# Autodesk Inventor assembly: Baugruppe1
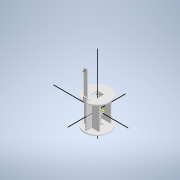
[picture p0: Inventor's stored thumbnail of the model, 180x180]
Saved by Autodesk Inventor 2022.2 (Build 262287010, 287A)
## iProperties
Created: 2023-12-11
Part Number: Baugruppe1
Document SubType Name: Assembly
Designer: ppovolni
Author: ppovolni
## Documents named in this file (13)
- D:\3_Local_Projekte\_PaperGitHub\MiniBumblebee_LowFieldMapping\2_Calibration\21_Hardware\213_CalibrationSolenoid_CAD\Slider\ASM_Slider_Inner.iam
- D:\3_Local_Projekte\_PaperGitHub\MiniBumblebee_LowFieldMapping\2_Calibration\21_Hardware\213_CalibrationSolenoid_CAD\Slider\Slider_Front.ipt
- D:\3_Local_Projekte\_PaperGitHub\MiniBumblebee_LowFieldMapping\2_Calibration\21_Hardware\213_CalibrationSolenoid_CAD\Slider\Conn_t15.ipt
- D:\3_Local_Projekte\_PaperGitHub\MiniBumblebee_LowFieldMapping\2_Calibration\21_Hardware\213_CalibrationSolenoid_CAD\Slider\Conn_t25.ipt
- D:\3_Local_Projekte\_PaperGitHub\MiniBumblebee_LowFieldMapping\2_Calibration\21_Hardware\213_CalibrationSolenoid_CAD\Slider\Conn_t60.ipt
- D:\3_Local_Projekte\_PaperGitHub\MiniBumblebee_LowFieldMapping\2_Calibration\21_Hardware\213_CalibrationSolenoid_CAD\Slider\Conn_t80.ipt
- D:\3_Local_Projekte\_PaperGitHub\MiniBumblebee_LowFieldMapping\2_Calibration\21_Hardware\213_CalibrationSolenoid_CAD\Slider\Slider_Angle.ipt
- D:\3_Local_Projekte\_PaperGitHub\MiniBumblebee_LowFieldMapping\2_Calibration\21_Hardware\213_CalibrationSolenoid_CAD\Slider\Screw-M6 x10.ipt
- D:\3_Local_Projekte\_PaperGitHub\MiniBumblebee_LowFieldMapping\2_Calibration\21_Hardware\213_CalibrationSolenoid_CAD\Slider\Screw-M6 x20.ipt.ipt
- D:\3_Local_Projekte\_PaperGitHub\MiniBumblebee_LowFieldMapping\2_Calibration\21_Hardware\213_CalibrationSolenoid_CAD\Slider\Slider_Angle_Distance_Holder.ipt
- D:\3_Local_Projekte\_PaperGitHub\MiniBumblebee_LowFieldMapping\2_Calibration\21_Hardware\213_CalibrationSolenoid_CAD\Slider\Hallsensor_Mounting\X-Axis\ASM_X-Axis.iam
- D:\3_Local_Projekte\_PaperGitHub\MiniBumblebee_LowFieldMapping\2_Calibration\21_Hardware\213_CalibrationSolenoid_CAD\Slider\Hallsensor_Mounting\Y-Axis\ASM_Y-Axis.iam
- D:\3_Local_Projekte\_PaperGitHub\MiniBumblebee_LowFieldMapping\2_Calibration\21_Hardware\213_CalibrationSolenoid_CAD\Slider\Hallsensor_Mounting\Z-Axis\ASM_Z-Axis.iam
## Components (13 placed, 12 different names)
1. Conn_t15:1 — Passend:4, Passend:9, Passend:10, Passend:13, Passend:24
2. Conn_t25:1 — Passend:3, Passend:11, Passend:12, Passend:26
3. Conn_t60:1 — Passend:2, Passend:7, Passend:8, Passend:25
4. Conn_t80:1 — Passend:1, Passend:5, Passend:6, Winkel:4, Passend:27, Passend:28, Passend:29, Passend:30, Passend:31, Passend:32, Passend:33, Passend:34
5. Slider_Angle:1 — Passend:16, Fluchtend:1, Passend:17, Passend:18, Passend:19, Winkel:3
6. DIN 912 - ersetzt durch DIN EN ISO 4762 M6 x 10:1 — Passend:20, Passend:23
7. DIN 912 - ersetzt durch DIN EN ISO 4762 M6 x 20:1 — Passend:21, Passend:22
8. Slider_Angle_Distance_Holder:1 — Passend:18, Passend:19, Winkel:3, Passend:20, Passend:21, Passend:22, Passend:23
9. ASM_X-Axis:1 [sub-assembly] — Winkel:4, Passend:27, Passend:28, Fluchtend:2, Fluchtend:3
10. ASM_Y-Axis:1 [sub-assembly] — Passend:29, Passend:30, Passend:31, Fluchtend:4, Fluchtend:5
11. ASM_Z-Axis:1 [sub-assembly] — Passend:32, Passend:33, Passend:34, Fluchtend:6, Fluchtend:7
12. Slider_Front:1 — Passend:1, Passend:2, Passend:3, Passend:4, Passend:5, Passend:6, Passend:7, Passend:8, Passend:9, Passend:10, Passend:11, Passend:12, Passend:16, Passend:17
13. Slider_Front:2 — Winkel:1
## Component patterns: (2 elements, first: Slider_Front:1)
## Relationships (42: Mate 32, Flush 7, Angle 3)
- Passend:1 [Mate]: Conn_t80:1 ↔ Slider_Front:1
- Passend:2 [Mate]: Conn_t60:1 ↔ Slider_Front:1
- Passend:3 [Mate]: Conn_t25:1 ↔ Slider_Front:1
- Passend:4 [Mate]: Conn_t15:1 ↔ Slider_Front:1
- Passend:5 [Mate] (0.1 mm): Conn_t80:1 ↔ Slider_Front:1
- Passend:6 [Mate] (0.1 mm): Conn_t80:1 ↔ Slider_Front:1
- Passend:7 [Mate] (0.1 mm): Conn_t60:1 ↔ Slider_Front:1
- Passend:8 [Mate] (0.1 mm): Conn_t60:1 ↔ Slider_Front:1
- Passend:9 [Mate]: Conn_t15:1 ↔ Slider_Front:1
- Passend:10 [Mate] (0.1 mm): Conn_t15:1 ↔ Slider_Front:1
- Passend:11 [Mate] (0.1 mm): Conn_t25:1 ↔ Slider_Front:1
- Passend:12 [Mate] (0.1 mm): Conn_t25:1 ↔ Slider_Front:1
- Passend:13 [Mate]: Conn_t15:1
- Winkel:1 [Angle] (0 deg): Slider_Front:2
- Passend:16 [Mate]: Slider_Angle:1 ↔ Slider_Front:1
- Fluchtend:1 [Flush] (10 mm): Slider_Angle:1
- Passend:17 [Mate]: Slider_Angle:1 ↔ Slider_Front:1
- Passend:18 [Mate]: Slider_Angle:1 ↔ Slider_Angle_Distance_Holder:1
- Passend:19 [Mate]: Slider_Angle:1 ↔ Slider_Angle_Distance_Holder:1
- Winkel:3 [Angle] (0 deg): Slider_Angle:1 ↔ Slider_Angle_Distance_Holder:1
- Passend:20 [Mate]: DIN 912 - ersetzt durch DIN EN ISO 4762 M6 x 10:1 ↔ Slider_Angle_Distance_Holder:1
- Passend:21 [Mate]: DIN 912 - ersetzt durch DIN EN ISO 4762 M6 x 20:1 ↔ Slider_Angle_Distance_Holder:1
- Passend:22 [Mate]: DIN 912 - ersetzt durch DIN EN ISO 4762 M6 x 20:1 ↔ Slider_Angle_Distance_Holder:1
- Passend:23 [Mate]: DIN 912 - ersetzt durch DIN EN ISO 4762 M6 x 10:1 ↔ Slider_Angle_Distance_Holder:1
- Passend:24 [Mate]: Conn_t15:1
- Passend:25 [Mate]: Conn_t60:1
- Passend:26 [Mate]: Conn_t25:1
- Winkel:4 [Angle] (0 deg): Conn_t80:1 ↔ ASM_X-Axis:1
- Passend:27 [Mate]: Conn_t80:1 ↔ ASM_X-Axis:1
- Passend:28 [Mate]: Conn_t80:1 ↔ ASM_X-Axis:1
- Fluchtend:2 [Flush]: ASM_X-Axis:1
- Fluchtend:3 [Flush]: ASM_X-Axis:1
- Passend:29 [Mate]: Conn_t80:1 ↔ ASM_Y-Axis:1
- Passend:30 [Mate]: Conn_t80:1 ↔ ASM_Y-Axis:1
- Passend:31 [Mate]: Conn_t80:1 ↔ ASM_Y-Axis:1
- Fluchtend:4 [Flush]: ASM_Y-Axis:1
- Fluchtend:5 [Flush]: ASM_Y-Axis:1
- Passend:32 [Mate]: Conn_t80:1 ↔ ASM_Z-Axis:1
- Passend:33 [Mate]: Conn_t80:1 ↔ ASM_Z-Axis:1
- Passend:34 [Mate]: Conn_t80:1 ↔ ASM_Z-Axis:1
- Fluchtend:6 [Flush]: ASM_Z-Axis:1
- Fluchtend:7 [Flush]: ASM_Z-Axis:1
